# Autodesk Inventor assembly: BodyV4_Left
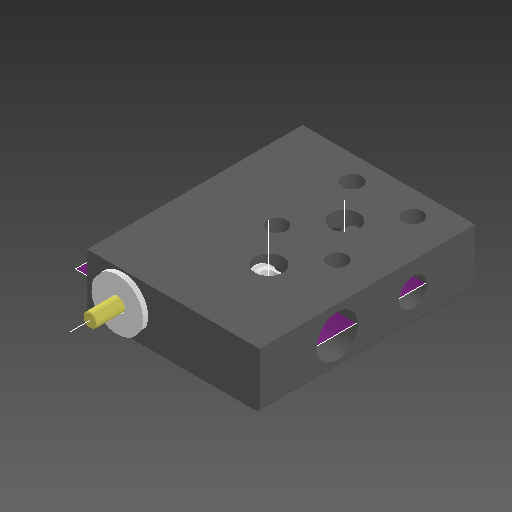
[picture p0: Inventor's stored thumbnail of the model, 512x512]
Saved by Autodesk Inventor 2021 (Build 250183000, 183)
## iProperties
Created: 2024-03-17
Part Number: BodyV4_Left
Document SubType Name: Assembly
Designer: top10
Author: top10
## Documents named in this file (4)
- D:\Files\Graduation Project\V4_manfoulid\Workspaces\Workspace\Left\BodyV4_Left.iam
- D:\Files\Graduation Project\V4_manfoulid\Workspaces\Workspace\Left\Val_BodV4_Left.ipt
- D:\Files\Graduation Project\V4_manfoulid\Workspaces\Workspace\R_nozzle\Left\rotarynozzle_Left3.iam
- D:\Files\Graduation Project\V4_manfoulid\Workspaces\Workspace\Left\CheckBall_Left.iam
## Components (3 placed, 3 different names)
1. Val_BodV4_Left:1 — Flush:3, Flush:2, Flush:1, Mate:1, Mate:3, Mate:2, Mate:6, Mate:4
2. rotarynozzle_Left3:1 [sub-assembly] — Mate:1, Mate:3, Mate:2
3. CheckBall_Left:1 [sub-assembly] — Mate:6, Mate:4
## Relationships (8: Mate 5, Flush 3)
- Flush:3: Val_BodV4_Left:1
- Flush:2: Val_BodV4_Left:1
- Flush:1: Val_BodV4_Left:1
- Mate:1 (-20 mm): Val_BodV4_Left:1 ↔ rotarynozzle_Left3:1
- Mate:3: Val_BodV4_Left:1 ↔ rotarynozzle_Left3:1
- Mate:2: Val_BodV4_Left:1 ↔ rotarynozzle_Left3:1
- Mate:6: Val_BodV4_Left:1 ↔ CheckBall_Left:1
- Mate:4: Val_BodV4_Left:1 ↔ CheckBall_Left:1
